# Autodesk Inventor assembly: Cuvette-rack
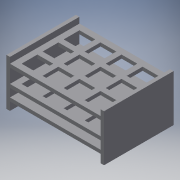
[picture p0: Inventor's stored thumbnail of the model, 180x180]
Saved by Autodesk Inventor 2018 (Build 220112000, 112)
## iProperties
Created: 2017-10-30
Part Number: Cuvette-rack
Document SubType Name: Assembly
Designer: xl0
Author: xl0
## Documents named in this file (6)
- E:\Alex\koi\Cuvette-rack\Parts\Cuvette-rack.iam
- E:\Alex\koi\Cuvette-rack\Parts\Top.ipt
- E:\Alex\koi\Cuvette-rack\Parts\Side.ipt
- E:\Alex\koi\Cuvette-rack\Parts\Bottom.ipt
- E:\Alex\koi\common\objects\clipboard\Clipboard.iam
- E:\Alex\koi\common\objects\Cuvette.ipt
## Components (8 placed, 5 different names)
1. Top:1 — Flush:1, Flush:2, Flush:3, Flush:4, Flush:5, Mate:2, Mate:7, Mate:8, Mate:9, Mate:10
2. Top:2 — Flush:4, Flush:5, Flush:6, Mate:3
3. Bottom:1 — Flush:7, Mate:1, Mate:5, Mate:6
4. Side:1 — Flush:1
5. Side:2 — Mate:1, Mate:2, Mate:3, Mate:4
6. Clipboard:1 [sub-assembly] — Mate:4
7. Cuvette:1 — Mate:5, Mate:7, Mate:8
8. Cuvette:2 — Mate:6, Mate:9, Mate:10
## Relationships (17: Mate 10, Flush 7)
- Flush:1: Top:1 ↔ Side:1
- Flush:2 (15 mm): Top:1
- Flush:3 (25 mm): Top:1
- Flush:4: Top:1 ↔ Top:2
- Flush:5: Top:1 ↔ Top:2
- Flush:6: Top:2
- Flush:7: Bottom:1
- Mate:1: Bottom:1 ↔ Side:2
- Mate:2: Top:1 ↔ Side:2
- Mate:3: Top:2 ↔ Side:2
- Mate:4: Side:2 ↔ Clipboard:1
- Mate:5: Bottom:1 ↔ Cuvette:1
- Mate:6: Bottom:1 ↔ Cuvette:2
- Mate:7 (0.5 mm): Top:1 ↔ Cuvette:1
- Mate:8 (0.5 mm): Top:1 ↔ Cuvette:1
- Mate:9 (0.5 mm): Top:1 ↔ Cuvette:2
- Mate:10 (0.5 mm): Top:1 ↔ Cuvette:2
